# Autodesk Inventor assembly: RearGearboxAssembly
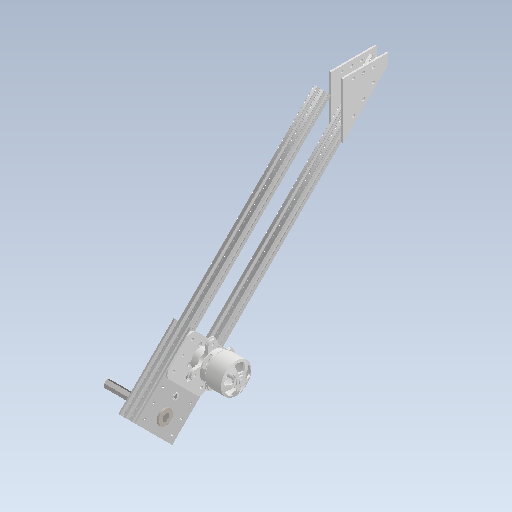
[picture p0: Inventor's stored thumbnail of the model, 512x512]
Saved by Autodesk Inventor 2023 (Build 270158000, 158)
## iProperties
Created: 2023-02-14
Part Number: RearGearboxAssembly
Document SubType Name: Assembly
Designer: Dave
Author: Dave
## Documents named in this file (6)
- C:\Users\Dave\Documents\GitHub\BehrendURCMechanical\CAD\Chassis\GearBox\Final Gears and Assemblies\RearGearboxAssembly.iam
- C:\Users\Dave\Documents\GitHub\BehrendURCMechanical\CAD\Chassis\GearBox\Final Gears and Assemblies\Gearbox Assembly.iam
- C:\Users\Dave\Documents\GitHub\BehrendURCMechanical\CAD\Chassis\CH-1-01-FrontKneeJoint.ipt
- C:\Users\Dave\Documents\GitHub\BehrendURCMechanical\CAD\Chassis\CH-1-01-20x20 Channel.ipt
- C:\Users\Dave\Documents\GitHub\BehrendURCMechanical\CAD\Chassis\CH-1-01-20x20 Channel\CH-1-01-20x20 Channel-604.ipt
- C:\Users\Dave\Documents\GitHub\BehrendURCMechanical\CAD\Chassis\CH-1-01-20x20 Channel\CH-1-01-20x20 Channel-528.ipt
## Components (5 placed, 4 different names)
1. Gearbox Assembly:1 [sub-assembly] — Angle:1, Flush:9, Mate:1, Flush:10, Flush:12, Mate:5, Flush:13, Flush:14
2. CH-1-01-FrontKneeJoint:1 — Flush:7, Flush:8, Flush:11, Mate:3
3. CH-1-01-FrontKneeJoint:2 — Flush:7, Flush:8, Mate:2, Mate:4
4. CH-1-01-20x20 Channel-604:1 — Flush:9, Mate:1, Flush:10, Flush:11, Mate:2, Mate:3, Mate:4
5. CH-1-01-20x20 Channel-528:2 — Flush:12, Mate:5, Flush:13, Flush:14
## Relationships (14: Flush 8, Mate 5, Angle 1)
- Angle:1 (45 deg): Gearbox Assembly:1
- Flush:7: CH-1-01-FrontKneeJoint:1 ↔ CH-1-01-FrontKneeJoint:2
- Flush:8: CH-1-01-FrontKneeJoint:1 ↔ CH-1-01-FrontKneeJoint:2
- Flush:9: Gearbox Assembly:1 ↔ CH-1-01-20x20 Channel-604:1
- Mate:1 (3.3 mm): Gearbox Assembly:1 ↔ CH-1-01-20x20 Channel-604:1
- Flush:10 (2.6924 mm): Gearbox Assembly:1 ↔ CH-1-01-20x20 Channel-604:1
- Flush:11: CH-1-01-FrontKneeJoint:1 ↔ CH-1-01-20x20 Channel-604:1
- Mate:2: CH-1-01-FrontKneeJoint:2 ↔ CH-1-01-20x20 Channel-604:1
- Mate:3: CH-1-01-FrontKneeJoint:1 ↔ CH-1-01-20x20 Channel-604:1
- Mate:4: CH-1-01-FrontKneeJoint:2 ↔ CH-1-01-20x20 Channel-604:1
- Flush:12: Gearbox Assembly:1 ↔ CH-1-01-20x20 Channel-528:2
- Mate:5 (3.3 mm): Gearbox Assembly:1 ↔ CH-1-01-20x20 Channel-528:2
- Flush:13 (2.6924 mm): Gearbox Assembly:1 ↔ CH-1-01-20x20 Channel-528:2
- Flush:14: Gearbox Assembly:1 ↔ CH-1-01-20x20 Channel-528:2
